# Autodesk Inventor assembly: Main_Assembly
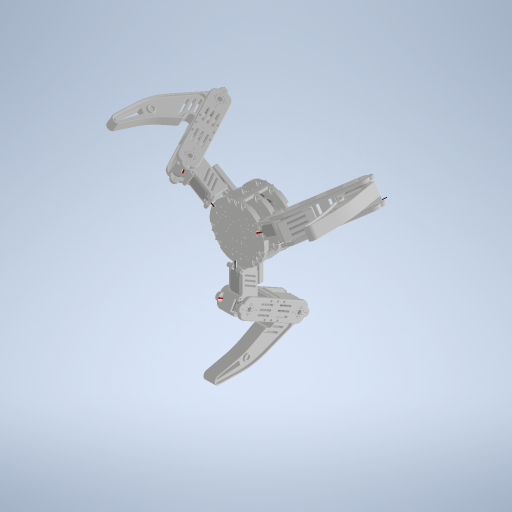
[picture p0: Inventor's stored thumbnail of the model, 512x512]
Saved by Autodesk Inventor 2023 (Build 270158000, 158)
## iProperties
Created: 2022-03-07
Part Number: Main_Assembly
Document SubType Name: Assembly
Designer: OEM
Author: OEM
## Documents named in this file (13)
- D:\Studia\Zebulon05\Zebulon05\Inventor_models\Main_Assembly.iam
- D:\Studia\Zebulon05\Zebulon05\Inventor_models\Body.ipt
- D:\Studia\Zebulon05\Zebulon05\Inventor_models\leg0.ipt
- D:\Studia\Zebulon05\Zebulon05\Inventor_models\Servo\HORN-D.ipt
- D:\Studia\Zebulon05\Zebulon05\Inventor_models\Servo\Case.ipt
- D:\Studia\Zebulon05\Zebulon05\Inventor_models\Leg1.ipt
- D:\Studia\Zebulon05\Zebulon05\Inventor_models\RPi Subs.ipt
- D:\Studia\Zebulon05\Zebulon05\Inventor_models\Spacer.ipt
- D:\Studia\Zebulon05\Zebulon05\Inventor_models\Leg2.ipt
- D:\Studia\Zebulon05\Zebulon05\Inventor_models\Leg3.ipt
- D:\Studia\Zebulon05\Zebulon05\Inventor_models\maestro_Subs.ipt
- D:\Studia\Zebulon05\Zebulon05\Inventor_models\step_down_Suba.ipt
- C:\Users\OEM\Documents\Inventor\Content Center Files\R2020\en-US\AS 1112 (2)\AS 1112 - M2  Type 5.ipt
## Components (49 placed, 17 different names)
1. Bod_lvl_plus1 — Mate:24, Mate:25, Mate:26, Mate:35, Mate:36, Mate:39, Mate:153, Mate:156, Mate:157, Mate:158, Mate:159, Mate:160, Mate:161, Mate:162, Mate:163, Mate:164, Mate:165, Mate:166, Mate:168
2. Body_lvl_Rpi — Mate:15, Mate:16, Mate:17, Mate:21, Mate:22, Mate:23, Mate:27, Mate:28, Mate:29, Mate:34, Mate:38, Mate:41, Mate:44, Mate:45, Mate:46, Mate:47, Mate:131, Mate:132, Mate:133, Mate:134, Mate:135, Mate:136
3. Body_lvl_FPGA — Mate:30, Mate:31, Mate:32, Mate:33, Mate:37, Mate:40, Mate:42, Mate:43
4. leg_part_0 — Mate:15, Mate:16, Mate:17, Mate:50
5. Leg_part_1 — Mate:51, Mate:53, Mate:54, Mate:56
6. Leg_part_3 — Mate:140, Mate:141
7. leg0:2 — Mate:131, Mate:132, Mate:133
8. HORN-D:4
9. Case:7
10. Leg1:2
11. Case:8
12. HORN-D:5
13. Leg2:5
14. Leg2:6
15. HORN-D:6
16. Case:9 — Mate:137, Mate:138, Mate:139
17. Leg3:2 — Mate:137, Mate:138, Mate:139
18. leg0:3 — Mate:134, Mate:135, Mate:136, Mate:149
19. HORN-D:7
20. Case:10 — Mate:149, Mate:150
21. Leg1:3 — Mate:148, Mate:150
22. Case:11 — Mate:148
23. HORN-D:8
24. Leg2:7 — Cylindrical:1, Mate:151, Mate:152
25. Leg2:8 — Mate:151, Mate:152
26. HORN-D:9
27. Case:12 — Mate:145, Mate:146, Mate:147, Cylindrical:1
28. Leg3:3 — Mate:145, Mate:146, Mate:147
29. Spacer:8 — Mate:33, Mate:34, Mate:37
30. Spacer:7 — Mate:39, Mate:41, Mate:44
31. Spacer:6 — Mate:35, Mate:36, Mate:38
32. Spacer:5 — Mate:40, Mate:42, Mate:43
33. Spacer:3 — Mate:21, Mate:22, Mate:23, Mate:24, Mate:25, Mate:26
34. Spacer:4 — Mate:27, Mate:28, Mate:29, Mate:30, Mate:31, Mate:32
35. step_down_Suba:2 — Mate:156, Mate:157, Mate:158
36. step_down_Suba:3 — Mate:161, Mate:162, Mate:163
37. AS 1112 (2) - Metric M2  Type 5:1 — Mate:166, Mate:167
38. AS 1112 (2) - Metric M2  Type 5:2 — Mate:168
39. step_down_Suba:1 — Mate:153, Mate:159, Mate:160
40. maestro_Subs:1 — Mate:164, Mate:165, Mate:167
41. RPi Subs:1 — Mate:45, Mate:46, Mate:47
42. Case:3 — Mate:8, Mate:9, Mate:51, Mate:53
43. HORN-D:1 — Mate:8, Mate:9, Mate:50
44. HORN-D:2 — Mate:13, Mate:60
45. Case:5 — Mate:13, Mate:54, Mate:56
46. Leg2:4 — Mate:63
47. Leg2:2 — Mate:60, Mate:63, Mate:74
48. Case:6 — Mate:67, Mate:68, Mate:140, Mate:141
49. HORN-D:3 — Mate:67, Mate:68, Mate:74
## Relationships (107: Mate 106, CylindricalJoint 1)
- Mate:8: Case:3 ↔ HORN-D:1
- Mate:9: Case:3 ↔ HORN-D:1
- Mate:13: HORN-D:2 ↔ Case:5
- Mate:15: Body_lvl_Rpi ↔ leg_part_0
- Mate:16: Body_lvl_Rpi ↔ leg_part_0
- Mate:17: Body_lvl_Rpi ↔ leg_part_0
- Mate:21: Body_lvl_Rpi ↔ Spacer:3
- Mate:22: Body_lvl_Rpi ↔ Spacer:3
- Mate:23: Body_lvl_Rpi ↔ Spacer:3
- Mate:24: Bod_lvl_plus1 ↔ Spacer:3
- Mate:25: Bod_lvl_plus1 ↔ Spacer:3
- Mate:26: Bod_lvl_plus1 ↔ Spacer:3
- Mate:27: Body_lvl_Rpi ↔ Spacer:4
- Mate:28: Body_lvl_Rpi ↔ Spacer:4
- Mate:29: Body_lvl_Rpi ↔ Spacer:4
- Mate:30: Body_lvl_FPGA ↔ Spacer:4
- Mate:31: Body_lvl_FPGA ↔ Spacer:4
- Mate:32: Body_lvl_FPGA ↔ Spacer:4
- Mate:33: Body_lvl_FPGA ↔ Spacer:8
- Mate:34: Body_lvl_Rpi ↔ Spacer:8
- Mate:35: Bod_lvl_plus1 ↔ Spacer:6
- Mate:36: Bod_lvl_plus1 ↔ Spacer:6
- Mate:37: Body_lvl_FPGA ↔ Spacer:8
- Mate:38: Body_lvl_Rpi ↔ Spacer:6
- Mate:39: Bod_lvl_plus1 ↔ Spacer:7
- Mate:40: Body_lvl_FPGA ↔ Spacer:5
- Mate:41: Body_lvl_Rpi ↔ Spacer:7
- Mate:42: Body_lvl_FPGA ↔ Spacer:5
- Mate:43: Body_lvl_FPGA ↔ Spacer:5
- Mate:44: Body_lvl_Rpi ↔ Spacer:7
- Mate:45: Body_lvl_Rpi ↔ RPi Subs:1
- Mate:46: Body_lvl_Rpi ↔ RPi Subs:1
- Mate:47: Body_lvl_Rpi ↔ RPi Subs:1
- Mate:50: leg_part_0 ↔ HORN-D:1
- Mate:51: Leg_part_1 ↔ Case:3
- Mate:53: Leg_part_1 ↔ Case:3
- Mate:54: Leg_part_1 ↔ Case:5
- Mate:56: Leg_part_1 ↔ Case:5
- Mate:60: HORN-D:2 ↔ Leg2:2
- Mate:63: Leg2:4 ↔ Leg2:2
- Mate:67: Case:6 ↔ HORN-D:3
- Mate:68: Case:6 ↔ HORN-D:3
- Mate:74: Leg2:2 ↔ HORN-D:3
- [Mate]: HORN-D:4 ↔ Case:7
- [Mate]: HORN-D:4 ↔ Case:7
- [Mate]: Case:8 ↔ HORN-D:5
- [Mate]: Case:8 ↔ HORN-D:5
- [Mate]: leg0:2 ↔ HORN-D:4
- [Mate]: Case:7 ↔ Leg1:2
- [Mate]: Case:7 ↔ Leg1:2
- [Mate]: Leg1:2 ↔ Case:8
- [Mate]: Leg1:2 ↔ Case:8
- [Mate]: Case:8 ↔ Leg2:5
- [Mate]: HORN-D:5 ↔ Leg2:5
- [Mate]: Leg2:5 ↔ Leg2:6
- [Mate]: HORN-D:6 ↔ Case:9
- [Mate]: HORN-D:6 ↔ Case:9
- [Mate]: Leg2:5 ↔ HORN-D:6
- [Mate]: HORN-D:7 ↔ Case:10
- [Mate]: HORN-D:7 ↔ Case:10
- [Mate]: Case:11 ↔ HORN-D:8
- [Mate]: Case:11 ↔ HORN-D:8
- [Mate]: leg0:3 ↔ HORN-D:7
- [Mate]: Case:10 ↔ Leg1:3
- [Mate]: Case:10 ↔ Leg1:3
- [Mate]: Leg1:3 ↔ Case:11
- [Mate]: Leg1:3 ↔ Case:11
- [Mate]: Case:11 ↔ Leg2:7
- [Mate]: HORN-D:8 ↔ Leg2:7
- [Mate]: Leg2:7 ↔ Leg2:8
- [Mate]: HORN-D:9 ↔ Case:12
- [Mate]: HORN-D:9 ↔ Case:12
- [Mate]: Leg2:7 ↔ HORN-D:9
- Mate:131: Body_lvl_Rpi ↔ leg0:2
- Mate:132: Body_lvl_Rpi ↔ leg0:2
- Mate:133: Body_lvl_Rpi ↔ leg0:2
- Mate:134: Body_lvl_Rpi ↔ leg0:3
- Mate:135: Body_lvl_Rpi ↔ leg0:3
- Mate:136: Body_lvl_Rpi ↔ leg0:3
- Mate:137: Case:9 ↔ Leg3:2
- Mate:138: Case:9 ↔ Leg3:2
- Mate:139: Case:9 ↔ Leg3:2
- Mate:140: Leg_part_3 ↔ Case:6
- Mate:141: Leg_part_3 ↔ Case:6
- Mate:145: Case:12 ↔ Leg3:3
- Mate:146: Case:12 ↔ Leg3:3
- Mate:147: Case:12 ↔ Leg3:3
- Cylindrical:1: Leg2:7 ↔ Case:12
- Mate:148: Leg1:3 ↔ Case:11
- Mate:149: leg0:3 ↔ Case:10
- Mate:150: Case:10 ↔ Leg1:3
- Mate:151: Leg2:7 ↔ Leg2:8
- Mate:152: Leg2:7 ↔ Leg2:8
- Mate:153: Bod_lvl_plus1 ↔ step_down_Suba:1
- Mate:156: Bod_lvl_plus1 ↔ step_down_Suba:2
- Mate:157: Bod_lvl_plus1 ↔ step_down_Suba:2
- Mate:158: Bod_lvl_plus1 ↔ step_down_Suba:2
- Mate:159: Bod_lvl_plus1 ↔ step_down_Suba:1
- Mate:160: Bod_lvl_plus1 ↔ step_down_Suba:1
- Mate:161: Bod_lvl_plus1 ↔ step_down_Suba:3
- Mate:162: Bod_lvl_plus1 ↔ step_down_Suba:3
- Mate:163: Bod_lvl_plus1 ↔ step_down_Suba:3
- Mate:164: Bod_lvl_plus1 ↔ maestro_Subs:1
- Mate:165: Bod_lvl_plus1 ↔ maestro_Subs:1
- Mate:166: Bod_lvl_plus1 ↔ AS 1112 (2) - Metric M2  Type 5:1
- Mate:167: AS 1112 (2) - Metric M2  Type 5:1 ↔ maestro_Subs:1
- Mate:168: Bod_lvl_plus1 ↔ AS 1112 (2) - Metric M2  Type 5:2
## Named parameters: d102_d94 = 0 mm, d103_d95 = 0 mm, d109_d101 = 0 mm, d110_d21 = 0 mm, d113_d70 = 0 mm, d115_d72 = 0 mm, d116_d73 = 0 mm, d118_d75 = 0 mm, d119_d76 = 0 mm, d120_d79 = 0 mm, d123_d82 = 0 mm, d126_d85 = 0 mm, d127_d22 = 0 mm, d128_d26 = 0 mm, d129_d27 = 0 mm, d130_d94 = 0 mm, d131_d95 = 0 mm, d137_d101 = 0 mm, d138_d21 = 0 mm, d141_d70 = 0 mm, d143_d72 = 0 mm, d144_d73 = 0 mm, d146_d75 = 0 mm, d147_d76 = 0 mm, d148_d79 = 0 mm, d151_d82 = 0 mm, d154_d85 = 0 mm, d155_d22 = 0 mm, d156_d26 = 0 mm, d157_d27 = 0 mm
